# Autodesk Inventor assembly: Right-Arm-Base
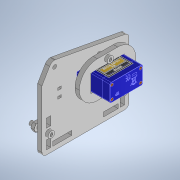
[picture p0: Inventor's stored thumbnail of the model, 180x180]
Saved by Autodesk Inventor 2022 (Build 260153000, 153)
## iProperties
Created: 2020-02-05
Part Number: Right-Arm-Base
Document SubType Name: Assembly
Designer: joshn
Author: joshn
Revision Number: NONE
## Documents named in this file (10)
- D:\Joshwin Emmanuel\Fab_accad\git_hub\Fab_Work\arm\step\part\Right-Arm-Base.iam
- D:\Joshwin Emmanuel\Fab_accad\git_hub\Fab_Work\arm\step\part\Right Arm Servo Plate.ipt
- D:\Joshwin Emmanuel\Fab_accad\git_hub\Fab_Work\arm\step\part\NONE_3.ipt
- D:\Joshwin Emmanuel\Fab_accad\git_hub\Fab_Work\arm\step\part\Schraube _ Zylinder - M3,0 x 8,0_1.ipt
- D:\Joshwin Emmanuel\Fab_accad\git_hub\Fab_Work\arm\step\part\Schraube _ Zylinder - M3,0 x 8,0_2.ipt
- D:\Joshwin Emmanuel\Fab_accad\git_hub\Fab_Work\arm\step\part\Zyl-Imbus M3x12.ipt
- D:\Joshwin Emmanuel\Fab_accad\git_hub\Fab_Work\arm\step\part\Zyl-Imbus M3x12_1.ipt
- D:\Joshwin Emmanuel\Fab_accad\git_hub\Fab_Work\arm\step\part\Mutter _  - M3,0 x 57,785_1.ipt
- D:\Joshwin Emmanuel\Fab_accad\git_hub\Fab_Work\arm\step\part\Mutter _  - M3,0 x 57,785_2.ipt
- D:\Joshwin Emmanuel\Fab_accad\git_hub\Fab_Work\arm\step\part\SG90 - Micro Servo 9g - Tower Pro.1.ipt
## Components (9 placed, 6 different names)
1. Right Arm Servo Plate — Mate:1, Mate:2
2. Right Servo Tower Pro SG90 — Mate:1, Mate:2, Mate:3
3. Servo Retainer — Mate:3
4. Schraube : Zylinder - M3,0 x 8,0
5. Schraube : Zylinder - M3,0 x 8,0:1
6. Zyl-Imbus M3x12
7. Zyl-Imbus M3x12:1
8. Mutter :  - M3,0 x 57,785
9. Mutter :  - M3,0 x 57,785:1
## Relationships (3: Mate 3)
- Mate:1: Right Arm Servo Plate ↔ Right Servo Tower Pro SG90
- Mate:2: Right Arm Servo Plate ↔ Right Servo Tower Pro SG90
- Mate:3: Right Servo Tower Pro SG90 ↔ Servo Retainer
